# Autodesk Inventor assembly: sliding_panel
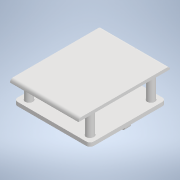
[picture p0: Inventor's stored thumbnail of the model, 180x180]
Saved by Autodesk Inventor 2022 (Build 260153000, 153)
## iProperties
Created: 2021-07-08
Part Number: sliding_panel
Document SubType Name: Assembly
Designer: fraaw
Author: fraaw
## Documents named in this file (4)
- C:\Users\fraaw\source\repos\fingerSense\CAD\sliding_panel.iam
- C:\Users\fraaw\source\repos\fingerSense\CAD\sliding_lifter.ipt
- C:\Users\fraaw\source\repos\fingerSense\CAD\sliding_platform.ipt
- C:\Users\fraaw\source\repos\fingerSense\CAD\sliding_support.ipt
## Components (3 placed, 3 different names)
1. sliding_support:1 — Mate:1, Mate:2, Mate:3, Mate:4, Mate:5
2. sliding_lifter:1 — Mate:1, Mate:2
3. sliding_platform:1 — Mate:3, Mate:4, Mate:5
## Relationships (5: Mate 5)
- Mate:1: sliding_support:1 ↔ sliding_lifter:1
- Mate:2: sliding_support:1 ↔ sliding_lifter:1
- Mate:3: sliding_support:1 ↔ sliding_platform:1
- Mate:4: sliding_support:1 ↔ sliding_platform:1
- Mate:5: sliding_support:1 ↔ sliding_platform:1
